# Autodesk Inventor assembly: Central Assembly
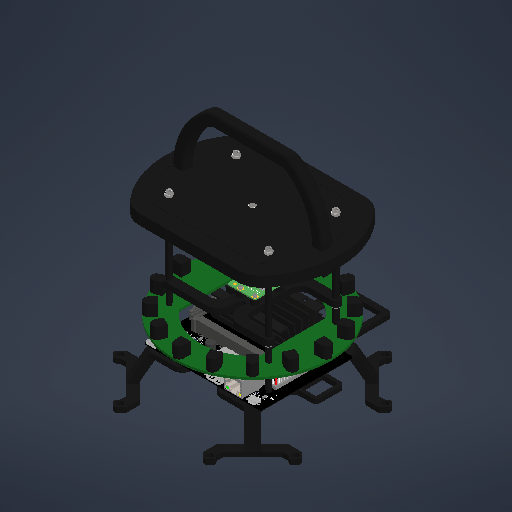
[picture p0: Inventor's stored thumbnail of the model, 512x512]
Saved by Autodesk Inventor 2026.1 (Build 301233020, 233B)
## iProperties
Created: 2026-02-20
Part Number: Central Assembly
Document SubType Name: Assembly
Designer: Bahaa
Mass: 260.821 g
Surface Area: 1859.36 cm^2
Volume: 215.571 cm^3
Density: 1.20991 g/cm^3
Author: Bahaa
## Documents named in this file (16)
- C:\Users\Bahaa\Nextcloud2\CAD\25-26\V1\Central Assembly.iam
- C:\Users\Bahaa\Documents\Inventor\Content Center Files\R2026\en-US\DIN 912\DIN 912 - M3 x 0,5 x 5 x 3,75.ipt
- C:\Users\Bahaa\Documents\Inventor\Content Center Files\R2026\en-US\DIN 985\DIN 985 - M3.ipt
- C:\Users\Bahaa\Documents\Inventor\Content Center Files\R2026\en-US\DIN 934\DIN 934 - M2,5 x 0,45.ipt
- C:\Users\Bahaa\Nextcloud2\CAD\25-26\V1\Rod Housing Jetson.ipt
- C:\Users\Bahaa\Nextcloud2\CAD\25-26\V1\Boards\IR Board.ipt
- C:\Users\Bahaa\Nextcloud2\CAD\25-26\V1\Rod Housing IR.ipt
- C:\Users\Bahaa\Nextcloud2\CAD\25-26\V1\Rod Housing Mirror.ipt
- C:\Users\Bahaa\Nextcloud2\CAD\25-26\V1\Parts\675_13541_batuu_dev_kit_top_ass_asm\675_13541_batuu_dev_kit_top_ass_asm.iam
- C:\Users\Bahaa\Nextcloud2\CAD\25-26\V1\Camera Bracket.ipt
- C:\Users\Bahaa\Nextcloud2\CAD\25-26\V1\Parts\Kamera.ipt
- C:\Users\Bahaa\Nextcloud2\CAD\25-26\V1\Top Cover.ipt
- C:\Users\Bahaa\Nextcloud2\CAD\25-26\V1\Mirror.ipt
- C:\Users\Bahaa\Documents\Inventor\Content Center Files\R2026\en-US\DIN 912\DIN 912 - M1,6 x 0,35 x 2,5 x 1,625.ipt
- C:\Users\Bahaa\Nextcloud2\CAD\25-26\V1\Handle.ipt
- C:\Users\Bahaa\Nextcloud2\CAD\25-26\V1\Center Hub neu.ipt
## Components (37 placed, 15 different names)
1. Camera Bracket:1 — Mate:56, Mate:59, Mate:60, Mate:61, Mate:62, Mate:63, Mate:64, Mate:65
2. Top Cover:1 — Mate:66, Mate:67, Mate:68, Insert:17, Mate:71, Mate:72, Mate:73, Insert:22, Insert:23, Insert:24, Insert:25
3. Mirror:1 — Mate:67, Mate:68
4. DIN 912 - replaced by DIN EN ISO 4762 M3 x 5:5 — Insert:17
5. DIN 912 - replaced by DIN EN ISO 4762 M1,6 x 2,5:1 — Insert:18
6. DIN 912 - replaced by DIN EN ISO 4762 M1,6 x 2,5:2 — Insert:19
7. DIN 912 - replaced by DIN EN ISO 4762 M1,6 x 2,5:3 — Insert:20
8. DIN 912 - replaced by DIN EN ISO 4762 M1,6 x 2,5:4 — Insert:21
9. Handle:1 — Mate:71, Mate:72, Mate:73
10. DIN 985 - replaced by DIN EN ISO 10511 M3:5 — Insert:22
11. DIN 985 - replaced by DIN EN ISO 10511 M3:6 — Insert:23
12. DIN 985 - replaced by DIN EN ISO 10511 M3:7 — Insert:24
13. DIN 985 - replaced by DIN EN ISO 10511 M3:8 — Insert:25
14. Center Hub neu:1 — Mate:74
15. Kamera:1 — Mate:59, Mate:60, Mate:61, Insert:18, Insert:19, Insert:20, Insert:21
16. 675_13541_batuu_dev_kit_top_ass_asm:1 [sub-assembly] — Mate:52, Mate:55, Mate:74
17. IR Board:1 — Mate:36, Mate:37, Mate:38, Mate:39, Mate:48, Mate:49, Mate:50, Mate:51
18. DIN 934 - replaced by DIN EN 24032/28673/28674 M2,5:5 — Insert:13
19. DIN 934 - replaced by DIN EN 24032/28673/28674 M2,5:6 — Insert:14
20. DIN 934 - replaced by DIN EN 24032/28673/28674 M2,5:7 — Insert:15, Mate:56
21. DIN 934 - replaced by DIN EN 24032/28673/28674 M2,5:8 — Insert:16
22. DIN 934 - replaced by DIN EN 24032/28673/28674 M2,5:1
23. DIN 934 - replaced by DIN EN 24032/28673/28674 M2,5:2
24. DIN 934 - replaced by DIN EN 24032/28673/28674 M2,5:3 — Mate:52
25. DIN 934 - replaced by DIN EN 24032/28673/28674 M2,5:4
26. Rod Housing Mirror:1 — Mate:64, Mate:66
27. Rod Housing Mirror:2 — Mate:62
28. Rod Housing Mirror:3 — Mate:65
29. Rod Housing Mirror:4 — Mate:63
30. Rod Housing IR:1 — Mate:39, Insert:13
31. Rod Housing IR:2 — Mate:38, Insert:15
32. Rod Housing IR:3 — Mate:37, Insert:16
33. Rod Housing IR:4 — Mate:36, Insert:14
34. Rod Housing Jetson:1 — Mate:49
35. Rod Housing Jetson:2 — Mate:51
36. Rod Housing Jetson:3 — Mate:50
37. Rod Housing Jetson:4 — Mate:48, Mate:55
## Relationships (38: Mate 25, Insert 13)
- Mate:36: IR Board:1 ↔ Rod Housing IR:4
- Mate:37: IR Board:1 ↔ Rod Housing IR:3
- Mate:38: IR Board:1 ↔ Rod Housing IR:2
- Mate:39: IR Board:1 ↔ Rod Housing IR:1
- Insert:13: DIN 934 - replaced by DIN EN 24032/28673/28674 M2,5:5 ↔ Rod Housing IR:1
- Insert:14: DIN 934 - replaced by DIN EN 24032/28673/28674 M2,5:6 ↔ Rod Housing IR:4
- Insert:15: DIN 934 - replaced by DIN EN 24032/28673/28674 M2,5:7 ↔ Rod Housing IR:2
- Insert:16: DIN 934 - replaced by DIN EN 24032/28673/28674 M2,5:8 ↔ Rod Housing IR:3
- Mate:48: IR Board:1 ↔ Rod Housing Jetson:4
- Mate:49: IR Board:1 ↔ Rod Housing Jetson:1
- Mate:50: IR Board:1 ↔ Rod Housing Jetson:3
- Mate:51: IR Board:1 ↔ Rod Housing Jetson:2
- Mate:52: 675_13541_batuu_dev_kit_top_ass_asm:1 ↔ DIN 934 - replaced by DIN EN 24032/28673/28674 M2,5:3
- Mate:55: 675_13541_batuu_dev_kit_top_ass_asm:1 ↔ Rod Housing Jetson:4
- Mate:56: Camera Bracket:1 ↔ DIN 934 - replaced by DIN EN 24032/28673/28674 M2,5:7
- Mate:59: Camera Bracket:1 ↔ Kamera:1
- Mate:60: Camera Bracket:1 ↔ Kamera:1
- Mate:61: Camera Bracket:1 ↔ Kamera:1
- Mate:62: Camera Bracket:1 ↔ Rod Housing Mirror:2
- Mate:63: Camera Bracket:1 ↔ Rod Housing Mirror:4
- Mate:64: Camera Bracket:1 ↔ Rod Housing Mirror:1
- Mate:65: Camera Bracket:1 ↔ Rod Housing Mirror:3
- Mate:66: Top Cover:1 ↔ Rod Housing Mirror:1
- Mate:67: Top Cover:1 ↔ Mirror:1
- Mate:68: Top Cover:1 ↔ Mirror:1
- Insert:17: Top Cover:1 ↔ DIN 912 - replaced by DIN EN ISO 4762 M3 x 5:5
- Insert:18: DIN 912 - replaced by DIN EN ISO 4762 M1,6 x 2,5:1 ↔ Kamera:1
- Insert:19: DIN 912 - replaced by DIN EN ISO 4762 M1,6 x 2,5:2 ↔ Kamera:1
- Insert:20: DIN 912 - replaced by DIN EN ISO 4762 M1,6 x 2,5:3 ↔ Kamera:1
- Insert:21: DIN 912 - replaced by DIN EN ISO 4762 M1,6 x 2,5:4 ↔ Kamera:1
- Mate:71: Top Cover:1 ↔ Handle:1
- Mate:72: Top Cover:1 ↔ Handle:1
- Mate:73: Top Cover:1 ↔ Handle:1
- Insert:22: Top Cover:1 ↔ DIN 985 - replaced by DIN EN ISO 10511 M3:5
- Insert:23: Top Cover:1 ↔ DIN 985 - replaced by DIN EN ISO 10511 M3:6
- Insert:24: Top Cover:1 ↔ DIN 985 - replaced by DIN EN ISO 10511 M3:7
- Insert:25: Top Cover:1 ↔ DIN 985 - replaced by DIN EN ISO 10511 M3:8
- Mate:74: Center Hub neu:1 ↔ 675_13541_batuu_dev_kit_top_ass_asm:1
